# Autodesk Inventor assembly: Tetrix_Chassis
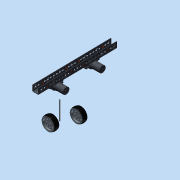
[picture p0: Inventor's stored thumbnail of the model, 180x180]
Saved by Autodesk Inventor 2015 (Build 190159000, 159)
## iProperties
Created: 2014-08-16
Part Number: Tetrix_Chassis
Document SubType Name: Assembly
Designer: Ashwin
Author: Ashwin
## Documents named in this file (7)
- C:\Users\Ashwin\Desktop\Robotics\CAD\drivetrain\drivetrain\Tetrix_Chassis.iam
- C:\Users\Ashwin\Desktop\Robotics\CAD\drivetrain\drivetrain\Imported Components\tetrix_739083_motor_2012\tetrix_739083_motor_2012.ipt
- C:\Users\Ashwin\Desktop\Robotics\CAD\drivetrain\drivetrain\Imported Components\tetrix_739089_2012\tetrix_739089_2012.ipt
- C:\Users\Ashwin\Desktop\Robotics\CAD\drivetrain\drivetrain\Imported Components\tetrix_739025_2012\tetrix_739025_2012.ipt
- C:\Users\Ashwin\Desktop\Robotics\CAD\drivetrain\drivetrain\Imported Components\tetrix_739069_2012\tetrix_739069_2012.ipt
- C:\Users\Ashwin\Desktop\Robotics\CAD\drivetrain\drivetrain\Imported Components\tetrix_739088_2013\tetrix_739088_2013.ipt
- C:\Users\Ashwin\Desktop\Robotics\CAD\drivetrain\drivetrain\Imported Components\tetrix_739091_2012\tetrix_739091_2012.ipt
## Components (16 placed, 6 different names)
1. tetrix_739025_2012:1
2. tetrix_739025_2012:2
3. tetrix_739069_2012:1 — Mate:2, Mate:8, Mate:9, Mate:10, Mate:12, Mate:13, Insert:1, Insert:3, Insert:4, Insert:5, Insert:6, Insert:7, Insert:8, Insert:9
4. tetrix_739083_motor_2012:1 — Mate:11, Flush:2
5. tetrix_739083_motor_2012:2 — Mate:14, Flush:3
6. tetrix_739089_2012:1 — Mate:2, Mate:12, Mate:13, Mate:14, Flush:3
7. tetrix_739089_2012:2 — Mate:8, Mate:9, Mate:10, Mate:11, Flush:2
8. tetrix_739088_2013:1
9. tetrix_739091_2012:1 — Insert:3
10. tetrix_739091_2012:2 — Insert:4
11. tetrix_739091_2012:3 — Insert:1
12. tetrix_739091_2012:4 — Insert:5
13. tetrix_739091_2012:5 — Insert:6
14. tetrix_739091_2012:6 — Insert:7
15. tetrix_739091_2012:7 — Insert:8
16. tetrix_739091_2012:8 — Insert:9
## Relationships (18: Mate 8, Insert 8, Flush 2)
- Mate:2: tetrix_739069_2012:1 ↔ tetrix_739089_2012:1
- Mate:8: tetrix_739069_2012:1 ↔ tetrix_739089_2012:2
- Mate:9: tetrix_739069_2012:1 ↔ tetrix_739089_2012:2
- Mate:10: tetrix_739069_2012:1 ↔ tetrix_739089_2012:2
- Mate:11: tetrix_739083_motor_2012:1 ↔ tetrix_739089_2012:2
- Flush:2: tetrix_739083_motor_2012:1 ↔ tetrix_739089_2012:2
- Mate:12: tetrix_739069_2012:1 ↔ tetrix_739089_2012:1
- Mate:13: tetrix_739069_2012:1 ↔ tetrix_739089_2012:1
- Mate:14: tetrix_739083_motor_2012:2 ↔ tetrix_739089_2012:1
- Flush:3: tetrix_739083_motor_2012:2 ↔ tetrix_739089_2012:1
- Insert:1: tetrix_739069_2012:1 ↔ tetrix_739091_2012:3
- Insert:3: tetrix_739069_2012:1 ↔ tetrix_739091_2012:1
- Insert:4: tetrix_739069_2012:1 ↔ tetrix_739091_2012:2
- Insert:5: tetrix_739069_2012:1 ↔ tetrix_739091_2012:4
- Insert:6: tetrix_739069_2012:1 ↔ tetrix_739091_2012:5
- Insert:7: tetrix_739069_2012:1 ↔ tetrix_739091_2012:6
- Insert:8: tetrix_739069_2012:1 ↔ tetrix_739091_2012:7
- Insert:9: tetrix_739069_2012:1 ↔ tetrix_739091_2012:8
